# Autodesk Inventor assembly: Base
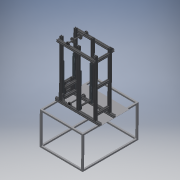
[picture p0: Inventor's stored thumbnail of the model, 180x180]
Saved by Autodesk Inventor 2016 (Build 200138000, 138)
## iProperties
Created: 2016-11-24
Part Number: Base
Material: 一般
Document SubType Name: Assembly
Designer: Daisuke
Author: Daisuke
## Documents named in this file (21)
- C:\Users\Daisuke\Documents\GitHub\CAD\Tomoato2016\Base\Base.iam
- C:\Users\Daisuke\Documents\GitHub\CAD\Tomoato2016\Base\HFS6-3030-750.ipt
- C:\Users\Daisuke\Documents\GitHub\CAD\Tomoato2016\Base\HFS6-3030-600.ipt
- C:\Users\Daisuke\Documents\GitHub\CAD\Tomoato2016\Base\HBLTF6-C_.ipt
- C:\Users\Daisuke\Documents\GitHub\CAD\Tomoato2016\Base\HFS6-3030-159.ipt
- C:\Users\Daisuke\Documents\GitHub\CAD\Tomoato2016\Base\HFS6-3030-500.ipt
- C:\Users\Daisuke\Documents\GitHub\CAD\Tomoato2016\Base\HBLFSNE6_.ipt
- C:\Users\Daisuke\Documents\GitHub\CAD\Tomoato2016\Base\SSRN3618.iam
- C:\Users\Daisuke\Documents\GitHub\CAD\Tomoato2016\Base\HFS6-3030-200.ipt
- C:\Users\Daisuke\Documents\GitHub\CAD\Tomoato2016\Base\HFS6-3030-140.ipt
- C:\Users\Daisuke\Documents\GitHub\CAD\Tomoato2016\Base\PBT12x.ipt
- C:\Users\Daisuke\Documents\GitHub\CAD\Tomoato2016\Base\HFS3-1515-30.ipt
- C:\Users\Daisuke\Documents\GitHub\CAD\Tomoato2016\Base\HFS3-1515-140.ipt
- C:\Users\Daisuke\Documents\GitHub\CAD\Tomoato2016\Base\NSFRQ15-241-F14-P12-T14-Q12-WKC60-C20-K60-E20_s.ipt
- C:\Users\Daisuke\Documents\GitHub\CAD\Tomoato2016\Base\NSFRQ15-181-F14-P12-T14-Q12-WKC30-C20-K30-E20_s.ipt
- C:\Users\Daisuke\Documents\GitHub\CAD\Tomoato2016\Base\KESS5-20.ipt
- C:\Users\Daisuke\Documents\GitHub\CAD\Tomoato2016\Base\SP25B32-N-15_b.ipt
- C:\Users\Daisuke\Documents\GitHub\CAD\Tomoato2016\Base\board.ipt
- C:\Users\Daisuke\Documents\GitHub\CAD\Tomoato2016\Base\frame710.ipt
- C:\Users\Daisuke\Documents\GitHub\CAD\Tomoato2016\Base\frame400.ipt
- C:\Users\Daisuke\Documents\GitHub\CAD\Tomoato2016\Base\frame577.ipt
## Components (52 placed, 20 different names)
1. HFS6-3030-750:1 — メイト:8, フラッシュ:9, フラッシュ:10, フラッシュ:32, フラッシュ:33, メイト:22, メイト:23, メイト:41, メイト:43
2. HFS6-3030-750:2 — メイト:9, フラッシュ:11, フラッシュ:12, メイト:21, メイト:24, フラッシュ:58
3. HFS6-3030-750:3 — メイト:10, フラッシュ:13, フラッシュ:14, メイト:11, フラッシュ:16, フラッシュ:18, メイト:13, フラッシュ:19, フラッシュ:20, メイト:14, フラッシュ:23, フラッシュ:24, メイト:18, フラッシュ:28, フラッシュ:29, フラッシュ:60, メイト:62, フラッシュ:61
4. HFS6-3030-750:4 — メイト:7, フラッシュ:7, フラッシュ:8, メイト:12, フラッシュ:15, フラッシュ:17, フラッシュ:21, フラッシュ:22, メイト:15, フラッシュ:25, フラッシュ:53, メイト:56
5. HFS6-3030-750:5 — メイト:6, フラッシュ:5, フラッシュ:6, フラッシュ:30, メイト:19, メイト:25, フラッシュ:56
6. HFS6-3030-750:6 — メイト:1, フラッシュ:1, メイト:3, メイト:4, フラッシュ:31, メイト:20, メイト:26, メイト:40, メイト:42
7. HFS6-3030-600:1 — メイト:8, フラッシュ:9, フラッシュ:10, メイト:9, フラッシュ:11, フラッシュ:12, メイト:10, フラッシュ:13, フラッシュ:14, メイト:37, フラッシュ:48
8. HFS6-3030-600:2 — メイト:1, フラッシュ:1, メイト:2, フラッシュ:2, フラッシュ:3, メイト:5, フラッシュ:4, メイト:6, フラッシュ:5, フラッシュ:6, メイト:7, フラッシュ:7, フラッシュ:8, メイト:36, フラッシュ:46, メイト:68, フラッシュ:62, フラッシュ:63
9. HBLTF6-C_:1 — メイト:2, フラッシュ:2, フラッシュ:3, メイト:3
10. HBLTF6-C_:2 — メイト:4, メイト:5, フラッシュ:4
11. HFS6-3030-159:1 — メイト:14, フラッシュ:23, フラッシュ:24
12. HFS6-3030-159:2 — メイト:11, メイト:12, フラッシュ:15, フラッシュ:16, フラッシュ:17, フラッシュ:18
13. HFS6-3030-159:3 — メイト:13, フラッシュ:19, フラッシュ:20, フラッシュ:21, フラッシュ:22
14. HFS6-3030-500:1 — メイト:18, フラッシュ:28, フラッシュ:29, メイト:38, フラッシュ:47
15. HFS6-3030-500:2 — メイト:15, フラッシュ:25, メイト:39, フラッシュ:45, フラッシュ:54, メイト:61
16. HBLFSNE6_:1 — フラッシュ:53, メイト:56, フラッシュ:54, メイト:61
17. SSRN3618:1 [sub-assembly] — フラッシュ:32, メイト:21, メイト:24, フラッシュ:57, メイト:58
18. SSRN3618:2 [sub-assembly] — フラッシュ:31, メイト:20, メイト:26, フラッシュ:35, メイト:29, メイト:30
19. SSRN3618:3 [sub-assembly] — フラッシュ:33, メイト:22, メイト:23, フラッシュ:34, メイト:27, メイト:28
20. SSRN3618:4 [sub-assembly] — フラッシュ:30, メイト:19, メイト:25, フラッシュ:55, メイト:57, メイト:59
21. HFS6-3030-200:1 — フラッシュ:34, メイト:27, メイト:28, フラッシュ:38, メイト:32, メイト:33, フラッシュ:39, フラッシュ:40, メイト:35, フラッシュ:43, フラッシュ:44
22. HFS6-3030-200:2 — フラッシュ:35, メイト:29, メイト:30, メイト:31, フラッシュ:36, フラッシュ:37, メイト:34, フラッシュ:41, フラッシュ:42
23. HFS6-3030-140:1 — メイト:31, フラッシュ:36, フラッシュ:37, フラッシュ:38, メイト:32
24. HFS6-3030-140:2 — メイト:33, フラッシュ:39, フラッシュ:40
25. HFS6-3030-140:3 — メイト:35, フラッシュ:41, フラッシュ:42
26. HFS6-3030-140:4 — メイト:34, フラッシュ:43, フラッシュ:44
27. PBT12x:1 — メイト:38, フラッシュ:47, メイト:43, 挿入:3
28. PBT12x:2 — メイト:37, フラッシュ:48, メイト:41
29. PBT12x:3 — メイト:39, フラッシュ:45, メイト:42, 挿入:2
30. PBT12x:4 — メイト:36, フラッシュ:46, メイト:40, 挿入:1
31. HFS3-1515-30:1 — フラッシュ:57, メイト:58, フラッシュ:58
32. HFS3-1515-30:2 — フラッシュ:55, メイト:57, フラッシュ:56, フラッシュ:59, メイト:60
33. HFS3-1515-140:1 — メイト:59, フラッシュ:59, メイト:60
34. HBLFSNE6_:2 — フラッシュ:60, メイト:62, フラッシュ:61
35. NSFRQ15-241-F14-P12-T14-Q12-WKC60-C20-K60-E20_s:1 — 挿入:2, 挿入:3, メイト:63, メイト:64, 正接:1, メイト:65, メイト:66, メイト:67
36. NSFRQ15-181-F14-P12-T14-Q12-WKC30-C20-K30-E20_s:1 — 挿入:1
37. KESS5-20:2 — メイト:63, メイト:64, 正接:1
38. SP25B32-N-15_b:2 — メイト:67
39. SP25B32-N-15_b:3 — メイト:65, メイト:66
40. board:1 — メイト:68, フラッシュ:62, フラッシュ:63, フラッシュ:86, メイト:80
41. frame710:1 — メイト:72, フラッシュ:70, フラッシュ:71, メイト:74, フラッシュ:74, フラッシュ:75
42. frame710:2 — メイト:73, フラッシュ:72, フラッシュ:73
43. frame710:3 — メイト:69, フラッシュ:64, フラッシュ:65
44. frame710:4 — メイト:70, フラッシュ:66, フラッシュ:67, メイト:71, フラッシュ:68, フラッシュ:69, フラッシュ:86, メイト:80
45. frame577:1 — メイト:72, フラッシュ:70, フラッシュ:71, メイト:73, フラッシュ:72, フラッシュ:73, メイト:79, フラッシュ:84, フラッシュ:85
46. frame577:2 — メイト:69, フラッシュ:64, フラッシュ:65, メイト:70, フラッシュ:66, フラッシュ:67, メイト:75, フラッシュ:76, フラッシュ:77, メイト:78, フラッシュ:82, フラッシュ:83
47. frame577:3 — メイト:74, フラッシュ:74, フラッシュ:75, メイト:76, フラッシュ:78, フラッシュ:79
48. frame577:4 — メイト:71, フラッシュ:68, フラッシュ:69, メイト:77, フラッシュ:80, フラッシュ:81
49. frame400:1 — メイト:75, フラッシュ:76, フラッシュ:77, メイト:76, フラッシュ:78, フラッシュ:79
50. frame400:2 — メイト:77, フラッシュ:80, フラッシュ:81
51. frame400:3 — メイト:78, フラッシュ:82, フラッシュ:83
52. frame400:4 — メイト:79, フラッシュ:84, フラッシュ:85
## Relationships (150: Flush 80, Mate 66, Insert 3, Tangent 1)
- メイト:1 [Mate]: HFS6-3030-750:6 ↔ HFS6-3030-600:2
- フラッシュ:1 [Flush]: HFS6-3030-750:6 ↔ HFS6-3030-600:2
- メイト:2 [Mate]: HFS6-3030-600:2 ↔ HBLTF6-C_:1
- フラッシュ:2 [Flush]: HFS6-3030-600:2 ↔ HBLTF6-C_:1
- フラッシュ:3 [Flush] (-5 mm): HFS6-3030-600:2 ↔ HBLTF6-C_:1
- メイト:3 [Mate]: HFS6-3030-750:6 ↔ HBLTF6-C_:1
- メイト:4 [Mate]: HFS6-3030-750:6 ↔ HBLTF6-C_:2
- メイト:5 [Mate]: HFS6-3030-600:2 ↔ HBLTF6-C_:2
- フラッシュ:4 [Flush] (5 mm): HFS6-3030-600:2 ↔ HBLTF6-C_:2
- メイト:6 [Mate]: HFS6-3030-750:5 ↔ HFS6-3030-600:2
- フラッシュ:5 [Flush]: HFS6-3030-750:5 ↔ HFS6-3030-600:2
- フラッシュ:6 [Flush] (285 mm): HFS6-3030-750:5 ↔ HFS6-3030-600:2
- メイト:7 [Mate]: HFS6-3030-750:4 ↔ HFS6-3030-600:2
- フラッシュ:7 [Flush]: HFS6-3030-750:4 ↔ HFS6-3030-600:2
- フラッシュ:8 [Flush] (55 mm): HFS6-3030-750:4 ↔ HFS6-3030-600:2
- メイト:8 [Mate]: HFS6-3030-750:1 ↔ HFS6-3030-600:1
- フラッシュ:9 [Flush]: HFS6-3030-750:1 ↔ HFS6-3030-600:1
- フラッシュ:10 [Flush] (55 mm): HFS6-3030-750:1 ↔ HFS6-3030-600:1
- メイト:9 [Mate]: HFS6-3030-750:2 ↔ HFS6-3030-600:1
- フラッシュ:11 [Flush]: HFS6-3030-750:2 ↔ HFS6-3030-600:1
- フラッシュ:12 [Flush] (285 mm): HFS6-3030-750:2 ↔ HFS6-3030-600:1
- メイト:10 [Mate]: HFS6-3030-750:3 ↔ HFS6-3030-600:1
- フラッシュ:13 [Flush]: HFS6-3030-750:3 ↔ HFS6-3030-600:1
- フラッシュ:14 [Flush] (55 mm): HFS6-3030-750:3 ↔ HFS6-3030-600:1
- メイト:11 [Mate]: HFS6-3030-750:3 ↔ HFS6-3030-159:2
- メイト:12 [Mate]: HFS6-3030-750:4 ↔ HFS6-3030-159:2
- フラッシュ:15 [Flush]: HFS6-3030-750:4 ↔ HFS6-3030-159:2
- フラッシュ:16 [Flush]: HFS6-3030-750:3 ↔ HFS6-3030-159:2
- フラッシュ:17 [Flush] (51 mm): HFS6-3030-750:4 ↔ HFS6-3030-159:2
- フラッシュ:18 [Flush] (51 mm): HFS6-3030-750:3 ↔ HFS6-3030-159:2
- メイト:13 [Mate]: HFS6-3030-750:3 ↔ HFS6-3030-159:3
- フラッシュ:19 [Flush]: HFS6-3030-750:3 ↔ HFS6-3030-159:3
- フラッシュ:20 [Flush] (51 mm): HFS6-3030-750:3 ↔ HFS6-3030-159:3
- フラッシュ:21 [Flush]: HFS6-3030-750:4 ↔ HFS6-3030-159:3
- フラッシュ:22 [Flush] (51 mm): HFS6-3030-750:4 ↔ HFS6-3030-159:3
- メイト:14 [Mate]: HFS6-3030-750:3 ↔ HFS6-3030-159:1
- フラッシュ:23 [Flush]: HFS6-3030-750:3 ↔ HFS6-3030-159:1
- フラッシュ:24 [Flush] (360 mm): HFS6-3030-750:3 ↔ HFS6-3030-159:1
- メイト:15 [Mate]: HFS6-3030-750:4 ↔ HFS6-3030-500:2
- フラッシュ:25 [Flush]: HFS6-3030-750:4 ↔ HFS6-3030-500:2
- メイト:18 [Mate]: HFS6-3030-750:3 ↔ HFS6-3030-500:1
- フラッシュ:28 [Flush]: HFS6-3030-750:3 ↔ HFS6-3030-500:1
- フラッシュ:29 [Flush] (-30 mm): HFS6-3030-750:3 ↔ HFS6-3030-500:1
- フラッシュ:30 [Flush]: HFS6-3030-750:5 ↔ SSRN3618:4
- メイト:19 [Mate]: HFS6-3030-750:5 ↔ SSRN3618:4
- フラッシュ:31 [Flush]: HFS6-3030-750:6 ↔ SSRN3618:2
- メイト:20 [Mate]: HFS6-3030-750:6 ↔ SSRN3618:2
- フラッシュ:32 [Flush]: HFS6-3030-750:1 ↔ SSRN3618:1
- メイト:21 [Mate]: HFS6-3030-750:2 ↔ SSRN3618:1
- フラッシュ:33 [Flush]: HFS6-3030-750:1 ↔ SSRN3618:3
- メイト:22 [Mate]: HFS6-3030-750:1 ↔ SSRN3618:3
- メイト:23 [Mate]: HFS6-3030-750:1 ↔ SSRN3618:3
- メイト:24 [Mate]: HFS6-3030-750:2 ↔ SSRN3618:1
- メイト:25 [Mate]: HFS6-3030-750:5 ↔ SSRN3618:4
- メイト:26 [Mate]: HFS6-3030-750:6 ↔ SSRN3618:2
- フラッシュ:34 [Flush]: SSRN3618:3 ↔ HFS6-3030-200:1
- メイト:27 [Mate]: SSRN3618:3 ↔ HFS6-3030-200:1
- メイト:28 [Mate]: SSRN3618:3 ↔ HFS6-3030-200:1
- フラッシュ:35 [Flush]: SSRN3618:2 ↔ HFS6-3030-200:2
- メイト:29 [Mate]: SSRN3618:2 ↔ HFS6-3030-200:2
- メイト:30 [Mate]: SSRN3618:2 ↔ HFS6-3030-200:2
- メイト:31 [Mate]: HFS6-3030-200:2 ↔ HFS6-3030-140:1
- フラッシュ:36 [Flush]: HFS6-3030-200:2 ↔ HFS6-3030-140:1
- フラッシュ:37 [Flush] (-30 mm): HFS6-3030-200:2 ↔ HFS6-3030-140:1
- フラッシュ:38 [Flush] (30 mm): HFS6-3030-200:1 ↔ HFS6-3030-140:1
- メイト:32 [Mate]: HFS6-3030-200:1 ↔ HFS6-3030-140:1
- メイト:33 [Mate]: HFS6-3030-200:1 ↔ HFS6-3030-140:2
- フラッシュ:39 [Flush]: HFS6-3030-200:1 ↔ HFS6-3030-140:2
- フラッシュ:40 [Flush] (30 mm): HFS6-3030-200:1 ↔ HFS6-3030-140:2
- メイト:34 [Mate]: HFS6-3030-200:2 ↔ HFS6-3030-140:4
- メイト:35 [Mate]: HFS6-3030-200:1 ↔ HFS6-3030-140:3
- フラッシュ:41 [Flush]: HFS6-3030-200:2 ↔ HFS6-3030-140:3
- フラッシュ:42 [Flush] (30 mm): HFS6-3030-200:2 ↔ HFS6-3030-140:3
- フラッシュ:43 [Flush]: HFS6-3030-200:1 ↔ HFS6-3030-140:4
- フラッシュ:44 [Flush] (30 mm): HFS6-3030-200:1 ↔ HFS6-3030-140:4
- メイト:36 [Mate]: HFS6-3030-600:2 ↔ PBT12x:4
- メイト:37 [Mate]: HFS6-3030-600:1 ↔ PBT12x:2
- メイト:38 [Mate]: HFS6-3030-500:1 ↔ PBT12x:1
- メイト:39 [Mate]: HFS6-3030-500:2 ↔ PBT12x:3
- フラッシュ:45 [Flush] (7 mm): HFS6-3030-500:2 ↔ PBT12x:3
- フラッシュ:46 [Flush] (7 mm): HFS6-3030-600:2 ↔ PBT12x:4
- フラッシュ:47 [Flush] (7 mm): HFS6-3030-500:1 ↔ PBT12x:1
- フラッシュ:48 [Flush] (7 mm): HFS6-3030-600:1 ↔ PBT12x:2
- メイト:40 [Mate] (64.5 mm): HFS6-3030-750:6 ↔ PBT12x:4
- メイト:41 [Mate] (64.5 mm): HFS6-3030-750:1 ↔ PBT12x:2
- メイト:42 [Mate] (64.5 mm): HFS6-3030-750:6 ↔ PBT12x:3
- メイト:43 [Mate] (64.5 mm): HFS6-3030-750:1 ↔ PBT12x:1
- フラッシュ:53 [Flush]: HFS6-3030-750:4 ↔ HBLFSNE6_:1
- メイト:56 [Mate]: HFS6-3030-750:4 ↔ HBLFSNE6_:1
- フラッシュ:54 [Flush] (5 mm): HFS6-3030-500:2 ↔ HBLFSNE6_:1
- フラッシュ:55 [Flush]: SSRN3618:4 ↔ HFS3-1515-30:2
- メイト:57 [Mate]: SSRN3618:4 ↔ HFS3-1515-30:2
- フラッシュ:56 [Flush] (5 mm): HFS6-3030-750:5 ↔ HFS3-1515-30:2
- フラッシュ:57 [Flush]: SSRN3618:1 ↔ HFS3-1515-30:1
- メイト:58 [Mate]: SSRN3618:1 ↔ HFS3-1515-30:1
- フラッシュ:58 [Flush] (5 mm): HFS6-3030-750:2 ↔ HFS3-1515-30:1
- メイト:59 [Mate]: SSRN3618:4 ↔ HFS3-1515-140:1
- フラッシュ:59 [Flush]: HFS3-1515-30:2 ↔ HFS3-1515-140:1
- メイト:60 [Mate]: HFS3-1515-30:2 ↔ HFS3-1515-140:1
- メイト:61 [Mate]: HFS6-3030-500:2 ↔ HBLFSNE6_:1
- フラッシュ:60 [Flush]: HFS6-3030-750:3 ↔ HBLFSNE6_:2
- メイト:62 [Mate]: HFS6-3030-750:3 ↔ HBLFSNE6_:2
- フラッシュ:61 [Flush] (-5 mm): HFS6-3030-750:3 ↔ HBLFSNE6_:2
- 挿入:1 [Insert]: PBT12x:4 ↔ NSFRQ15-181-F14-P12-T14-Q12-WKC30-C20-K30-E20_s:1
- 挿入:2 [Insert]: PBT12x:3 ↔ NSFRQ15-241-F14-P12-T14-Q12-WKC60-C20-K60-E20_s:1
- 挿入:3 [Insert]: PBT12x:1 ↔ NSFRQ15-241-F14-P12-T14-Q12-WKC60-C20-K60-E20_s:1
- メイト:63 [Mate]: NSFRQ15-241-F14-P12-T14-Q12-WKC60-C20-K60-E20_s:1 ↔ KESS5-20:2
- メイト:64 [Mate]: NSFRQ15-241-F14-P12-T14-Q12-WKC60-C20-K60-E20_s:1 ↔ KESS5-20:2
- 正接:1 [Tangent]: NSFRQ15-241-F14-P12-T14-Q12-WKC60-C20-K60-E20_s:1 ↔ KESS5-20:2
- メイト:65 [Mate]: NSFRQ15-241-F14-P12-T14-Q12-WKC60-C20-K60-E20_s:1 ↔ SP25B32-N-15_b:3
- メイト:66 [Mate]: NSFRQ15-241-F14-P12-T14-Q12-WKC60-C20-K60-E20_s:1 ↔ SP25B32-N-15_b:3
- メイト:67 [Mate]: NSFRQ15-241-F14-P12-T14-Q12-WKC60-C20-K60-E20_s:1 ↔ SP25B32-N-15_b:2
- メイト:68 [Mate]: HFS6-3030-600:2 ↔ board:1
- フラッシュ:62 [Flush]: HFS6-3030-600:2 ↔ board:1
- フラッシュ:63 [Flush]: HFS6-3030-600:2 ↔ board:1
- メイト:69 [Mate]: frame710:3 ↔ frame577:2
- フラッシュ:64 [Flush]: frame710:3 ↔ frame577:2
- フラッシュ:65 [Flush]: frame710:3 ↔ frame577:2
- メイト:70 [Mate]: frame710:4 ↔ frame577:2
- フラッシュ:66 [Flush]: frame710:4 ↔ frame577:2
- フラッシュ:67 [Flush]: frame710:4 ↔ frame577:2
- メイト:71 [Mate]: frame710:4 ↔ frame577:4
- フラッシュ:68 [Flush]: frame710:4 ↔ frame577:4
- フラッシュ:69 [Flush]: frame710:4 ↔ frame577:4
- メイト:72 [Mate]: frame710:1 ↔ frame577:1
- フラッシュ:70 [Flush]: frame710:1 ↔ frame577:1
- フラッシュ:71 [Flush]: frame710:1 ↔ frame577:1
- メイト:73 [Mate]: frame710:2 ↔ frame577:1
- フラッシュ:72 [Flush]: frame710:2 ↔ frame577:1
- フラッシュ:73 [Flush]: frame710:2 ↔ frame577:1
- メイト:74 [Mate]: frame710:1 ↔ frame577:3
- フラッシュ:74 [Flush]: frame710:1 ↔ frame577:3
- フラッシュ:75 [Flush]: frame710:1 ↔ frame577:3
- メイト:75 [Mate]: frame577:2 ↔ frame400:1
- フラッシュ:76 [Flush]: frame577:2 ↔ frame400:1
- フラッシュ:77 [Flush]: frame577:2 ↔ frame400:1
- メイト:76 [Mate]: frame577:3 ↔ frame400:1
- フラッシュ:78 [Flush]: frame577:3 ↔ frame400:1
- フラッシュ:79 [Flush]: frame577:3 ↔ frame400:1
- メイト:77 [Mate]: frame577:4 ↔ frame400:2
- フラッシュ:80 [Flush]: frame577:4 ↔ frame400:2
- フラッシュ:81 [Flush]: frame577:4 ↔ frame400:2
- メイト:78 [Mate]: frame577:2 ↔ frame400:3
- フラッシュ:82 [Flush]: frame577:2 ↔ frame400:3
- フラッシュ:83 [Flush]: frame577:2 ↔ frame400:3
- メイト:79 [Mate]: frame577:1 ↔ frame400:4
- フラッシュ:84 [Flush]: frame577:1 ↔ frame400:4
- フラッシュ:85 [Flush]: frame577:1 ↔ frame400:4
- フラッシュ:86 [Flush]: board:1 ↔ frame710:4
- メイト:80 [Mate]: board:1 ↔ frame710:4
